# Autodesk Inventor assembly: Bari Cart
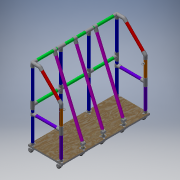
[picture p0: Inventor's stored thumbnail of the model, 180x180]
Saved by Autodesk Inventor 2018.2 (Build 222227000, 227)
## iProperties
Created: 2018-03-15
Part Number: Bari Cart
Document SubType Name: Assembly
Designer: owner
Author: owner
## Documents named in this file (20)
- Z:\The Pickle - 4 - Copy\Final Carts\Sax Cart\Bari Sax Cart.iam
- Z:\The Pickle - 4 - Copy\Final Carts\Sax Cart\Bari Plywood Base.ipt
- Z:\The Pickle - 4 - Copy\Final Carts\Stuff Used By All Carts\PVC Fittings (Formufit)\Wood Mount 1 Inch.ipt
- Z:\The Pickle - 4 - Copy\Final Carts\Stuff Used By All Carts\PVC Fittings (Formufit)\3-way 90 1 Inch.ipt
- Z:\The Pickle - 4 - Copy\Final Carts\Stuff Used By All Carts\PVC Fittings (Formufit)\45 Elbow 1 Inch.ipt
- Z:\The Pickle - 4 - Copy\Final Carts\Stuff Used By All Carts\PVC Fittings (Formufit)\Cross 1 Inch.ipt
- Z:\The Pickle - 4 - Copy\Final Carts\Stuff Used By All Carts\PVC Fittings (Formufit)\Formufit Pipe 1 Inch Flush Fittings.ipt
- Z:\The Pickle - 4 - Copy\Final Carts\Stuff Used By All Carts\PVC Fittings (Formufit)\Slip Tee 1 Inch.ipt
- Z:\The Pickle - 4 - Copy\Final Carts\Stuff Used By All Carts\PVC Fittings (Formufit)\Tee 1 Inch.ipt
- Z:\The Pickle - 4 - Copy\Final Carts\Sax Cart\Adjustable Elbow 1 Inch - Sax Angle.iam
- Z:\The Pickle - 4 - Copy\Final Carts\Sax Cart\Sax Pipe 1 (Tenor and Bari).ipt
- Z:\The Pickle - 4 - Copy\Final Carts\Sax Cart\Sax Pipe 2 (Tenor and Bari).ipt
- Z:\The Pickle - 4 - Copy\Final Carts\Sax Cart\Bari Sax Pipe 5.ipt
- Z:\The Pickle - 4 - Copy\Final Carts\Sax Cart\Bari Sax Pipe 4.ipt
- Z:\The Pickle - 4 - Copy\Final Carts\Sax Cart\Bari Sax Pipe 6.ipt
- Z:\The Pickle - 4 - Copy\Final Carts\Sax Cart\Bari Sax Pipe 7.ipt
- Z:\The Pickle - 4 - Copy\Final Carts\Sax Cart\Bari Sax Pipe OD - ID Adaptor.ipt
- Z:\The Pickle - 4 - Copy\Final Carts\Sax Cart\Bari Sax Wheel.ipt
- Z:\The Pickle - 4 - Copy\Final Carts\Sax Cart\Eyenut Screw.ipt
- Z:\The Pickle - 4 - Copy\Final Carts\Sax Cart\Eyenut.ipt
## Components (76 placed, 19 different names)
1. Bari Plywood Base:1 — Mate:1, Tangent:1, Tangent:2, Tangent:3, Mate:10, Mate:11, Mate:12, Flush:32, Flush:33, Flush:34, Mate:16, Tangent:4, Tangent:5, Flush:35
2. Wood Mount 1 Inch:1 — Mate:1, Tangent:1, Tangent:2, Tangent:3, Insert:1
3. Wood Mount 1 Inch:3 — Flush:3, Insert:6, Tangent:4
4. Wood Mount 1 Inch:4 — Flush:3, Flush:4, Insert:4, Tangent:5
5. Wood Mount 1 Inch:5 — Flush:5, Insert:3
6. Wood Mount 1 Inch:6 — Insert:2
7. Wood Mount 1 Inch:8 — Flush:4, Flush:5, Insert:5
8. 3-way 90 1 Inch:1 — Insert:18, Insert:21, Mate:8
9. 3-way 90 1 Inch:2 — Insert:35, Insert:37, Insert:39
10. 45 Elbow 1 Inch:1 — Insert:14, Mate:30
11. 45 Elbow 1 Inch:2 — Insert:42, Insert:43, Mate:27
12. 45 Elbow 1 Inch:3 — Insert:16, Insert:17
13. 45 Elbow 1 Inch:4 — Insert:40, Insert:41
14. Cross 1 Inch:1 — Insert:23, Insert:27, Insert:28
15. Cross 1 Inch:2 — Insert:30, Insert:31, Insert:33
16. Formufit Pipe 1 Inch Flush Fittings:1 — Insert:39, Insert:40
17. Formufit Pipe 1 Inch Flush Fittings:2 — Insert:17, Insert:18
18. Slip Tee 1 Inch:1 — Insert:12, Mate:2
19. Slip Tee 1 Inch:2 — Insert:47, Mate:3
20. Slip Tee 1 Inch:3 — Mate:6, Mate:9, Mate:15
21. Slip Tee 1 Inch:4 — Mate:5, Mate:7, Mate:9, Mate:14
22. Tee 1 Inch:1 — Insert:19, Insert:20, Insert:22
23. Tee 1 Inch:2 — Insert:36, Insert:38
24. Tee 1 Inch:3 — Insert:24, Insert:25, Insert:26
25. Tee 1 Inch:4 — Insert:29, Insert:32, Insert:34
26. Tee 1 Inch:5 — Insert:44, Insert:45, Insert:46, Mate:28
27. Tee 1 Inch:6 — Insert:10, Insert:11, Insert:13, Mate:31
28. Adjustable Elbow 1 Inch - Sax Angle:1 [sub-assembly] — Insert:53, Mate:15, Insert:56
29. Adjustable Elbow 1 Inch - Sax Angle:2 [sub-assembly] — Insert:51, Mate:13, Insert:54
30. Adjustable Elbow 1 Inch - Sax Angle:3 [sub-assembly] — Insert:52, Mate:14, Insert:55
31. Sax Pipe 1 (Tenor and Bari):1 — Insert:3, Insert:31
32. Sax Pipe 1 (Tenor and Bari):2 — Insert:4, Insert:38, Mate:3, Mate:23
33. Sax Pipe 1 (Tenor and Bari):3 — Insert:5, Insert:28
34. Sax Pipe 1 (Tenor and Bari):4 — Insert:20
35. Sax Pipe 1 (Tenor and Bari):5 — Insert:25
36. Sax Pipe 1 (Tenor and Bari):6 — Insert:32
37. Sax Pipe 1 (Tenor and Bari):7 — Insert:37, Mate:21, Mate:22
38. Sax Pipe 1 (Tenor and Bari):8 — Insert:2, Mate:2, Insert:19
39. Sax Pipe 2 (Tenor and Bari):1 — Insert:21, Insert:24, Mate:4
40. Sax Pipe 2 (Tenor and Bari):2 — Insert:26, Insert:29, Mate:5
41. Sax Pipe 2 (Tenor and Bari):3 — Insert:33, Insert:36
42. Sax Pipe 2 (Tenor and Bari):4 — Insert:34, Insert:35, Mate:6
43. Sax Pipe 2 (Tenor and Bari):5 — Insert:27, Insert:30
44. Sax Pipe 2 (Tenor and Bari):6 — Insert:22, Insert:23
45. Bari Sax Pipe 5:1 — Insert:11, Insert:12
46. Bari Sax Pipe 5:2 — Insert:46, Insert:47
47. Bari Sax Pipe 5:3 — Insert:1, Insert:10
48. Bari Sax Pipe 5:4 — Insert:6, Insert:45
49. Bari Sax Pipe 4:1 — Insert:54, Mate:17
50. Bari Sax Pipe 4:2 — Insert:55, Mate:18
51. Bari Sax Pipe 6:1 — Insert:16
52. Bari Sax Pipe 6:2 — Insert:41, Insert:42
53. Bari Sax Pipe 7:1 — Insert:13, Insert:14, Tangent:8, Tangent:9
54. Bari Sax Pipe 7:2 — Insert:43, Insert:44, Mate:20, Tangent:6, Tangent:7
55. Slip Tee 1 Inch:5 — Mate:4, Mate:7, Mate:8, Mate:13
56. Wood Mount 1 Inch:11 — Mate:10, Insert:50
57. Wood Mount 1 Inch:12 — Mate:11, Insert:49
58. Wood Mount 1 Inch:13 — Mate:12, Insert:48
59. Bari Sax Pipe OD - ID Adaptor:1 — Insert:48, Insert:53
60. Bari Sax Pipe OD - ID Adaptor:2 — Insert:50, Insert:51
61. Bari Sax Pipe OD - ID Adaptor:3 — Insert:49, Insert:52
62. Bari Sax Pipe 4:3 — Insert:56, Mate:19
63. Bari Sax Wheel:1 — Flush:6, Flush:10, Flush:15, Flush:22, Flush:32, Flush:33
64. Bari Sax Wheel:2 — Flush:6, Flush:7, Flush:11, Flush:16, Flush:22, Flush:23, Mate:17
65. Bari Sax Wheel:3 — Flush:7, Flush:8, Flush:12, Flush:17, Flush:23, Flush:24, Mate:18
66. Bari Sax Wheel:4 — Flush:8, Flush:9, Flush:13, Flush:18, Flush:24, Flush:25, Mate:19
67. Bari Sax Wheel:5 — Flush:9, Flush:19, Flush:25, Flush:35
68. Bari Sax Wheel:6 — Flush:14, Flush:19, Flush:27
69. Bari Sax Wheel:7 — Flush:13, Flush:14, Flush:18, Flush:26, Flush:27
70. Bari Sax Wheel:8 — Flush:12, Flush:17, Flush:21, Flush:26
71. Bari Sax Wheel:9 — Flush:11, Flush:16, Flush:20, Flush:21
72. Bari Sax Wheel:10 — Flush:10, Flush:15, Flush:20, Flush:34, Mate:16
73. Eyenut Screw:1 — Tangent:6, Mate:26, Mate:27, Mate:28
74. Eyenut:1 — Tangent:7, Mate:26
75. Eyenut Screw:2 — Mate:29, Tangent:9, Mate:30, Mate:31
76. Eyenut:2 — Mate:29, Tangent:8
## Relationships (121: Insert 52, Mate 31, Flush 29, Tangent 9)
- Flush:3: Wood Mount 1 Inch:3 ↔ Wood Mount 1 Inch:4
- Flush:4: Wood Mount 1 Inch:4 ↔ Wood Mount 1 Inch:8
- Flush:5: Wood Mount 1 Inch:5 ↔ Wood Mount 1 Inch:8
- Mate:1: Bari Plywood Base:1 ↔ Wood Mount 1 Inch:1
- Tangent:1: Bari Plywood Base:1 ↔ Wood Mount 1 Inch:1
- Tangent:2: Bari Plywood Base:1 ↔ Wood Mount 1 Inch:1
- Tangent:3: Bari Plywood Base:1 ↔ Wood Mount 1 Inch:1
- Insert:1: Wood Mount 1 Inch:1 ↔ Bari Sax Pipe 5:3
- Insert:2: Wood Mount 1 Inch:6 ↔ Sax Pipe 1 (Tenor and Bari):8
- Insert:3: Wood Mount 1 Inch:5 ↔ Sax Pipe 1 (Tenor and Bari):1
- Insert:4: Wood Mount 1 Inch:4 ↔ Sax Pipe 1 (Tenor and Bari):2
- Insert:5: Wood Mount 1 Inch:8 ↔ Sax Pipe 1 (Tenor and Bari):3
- Insert:6: Wood Mount 1 Inch:3 ↔ Bari Sax Pipe 5:4
- Insert:10: Tee 1 Inch:6 ↔ Bari Sax Pipe 5:3
- Insert:11: Tee 1 Inch:6 ↔ Bari Sax Pipe 5:1
- Insert:12: Slip Tee 1 Inch:1 ↔ Bari Sax Pipe 5:1
- Mate:2: Slip Tee 1 Inch:1 ↔ Sax Pipe 1 (Tenor and Bari):8
- Insert:13: Tee 1 Inch:6 ↔ Bari Sax Pipe 7:1
- Insert:14: 45 Elbow 1 Inch:1 ↔ Bari Sax Pipe 7:1
- Insert:16: 45 Elbow 1 Inch:3 ↔ Bari Sax Pipe 6:1
- Insert:17: 45 Elbow 1 Inch:3 ↔ Formufit Pipe 1 Inch Flush Fittings:2
- Insert:18: 3-way 90 1 Inch:1 ↔ Formufit Pipe 1 Inch Flush Fittings:2
- Insert:19: Tee 1 Inch:1 ↔ Sax Pipe 1 (Tenor and Bari):8
- Insert:20: Tee 1 Inch:1 ↔ Sax Pipe 1 (Tenor and Bari):4
- Insert:21: 3-way 90 1 Inch:1 ↔ Sax Pipe 2 (Tenor and Bari):1
- Insert:22: Tee 1 Inch:1 ↔ Sax Pipe 2 (Tenor and Bari):6
- Insert:23: Cross 1 Inch:1 ↔ Sax Pipe 2 (Tenor and Bari):6
- Insert:24: Tee 1 Inch:3 ↔ Sax Pipe 2 (Tenor and Bari):1
- Insert:25: Tee 1 Inch:3 ↔ Sax Pipe 1 (Tenor and Bari):5
- Insert:26: Tee 1 Inch:3 ↔ Sax Pipe 2 (Tenor and Bari):2
- Insert:27: Cross 1 Inch:1 ↔ Sax Pipe 2 (Tenor and Bari):5
- Insert:28: Cross 1 Inch:1 ↔ Sax Pipe 1 (Tenor and Bari):3
- Insert:29: Tee 1 Inch:4 ↔ Sax Pipe 2 (Tenor and Bari):2
- Insert:30: Cross 1 Inch:2 ↔ Sax Pipe 2 (Tenor and Bari):5
- Insert:31: Cross 1 Inch:2 ↔ Sax Pipe 1 (Tenor and Bari):1
- Insert:32: Tee 1 Inch:4 ↔ Sax Pipe 1 (Tenor and Bari):6
- Insert:33: Cross 1 Inch:2 ↔ Sax Pipe 2 (Tenor and Bari):3
- Insert:34: Tee 1 Inch:4 ↔ Sax Pipe 2 (Tenor and Bari):4
- Insert:35: 3-way 90 1 Inch:2 ↔ Sax Pipe 2 (Tenor and Bari):4
- Insert:36: Tee 1 Inch:2 ↔ Sax Pipe 2 (Tenor and Bari):3
- Insert:37: 3-way 90 1 Inch:2 ↔ Sax Pipe 1 (Tenor and Bari):7
- Insert:38: Tee 1 Inch:2 ↔ Sax Pipe 1 (Tenor and Bari):2
- Insert:39: 3-way 90 1 Inch:2 ↔ Formufit Pipe 1 Inch Flush Fittings:1
- Insert:40: 45 Elbow 1 Inch:4 ↔ Formufit Pipe 1 Inch Flush Fittings:1
- Insert:41: 45 Elbow 1 Inch:4 ↔ Bari Sax Pipe 6:2
- Insert:42: 45 Elbow 1 Inch:2 ↔ Bari Sax Pipe 6:2
- Insert:43: 45 Elbow 1 Inch:2 ↔ Bari Sax Pipe 7:2
- Insert:44: Tee 1 Inch:5 ↔ Bari Sax Pipe 7:2
- Insert:45: Tee 1 Inch:5 ↔ Bari Sax Pipe 5:4
- Insert:46: Tee 1 Inch:5 ↔ Bari Sax Pipe 5:2
- Insert:47: Slip Tee 1 Inch:2 ↔ Bari Sax Pipe 5:2
- Mate:3: Slip Tee 1 Inch:2 ↔ Sax Pipe 1 (Tenor and Bari):2
- Mate:4: Sax Pipe 2 (Tenor and Bari):1 ↔ Slip Tee 1 Inch:5
- Mate:5: Slip Tee 1 Inch:4 ↔ Sax Pipe 2 (Tenor and Bari):2
- Mate:6: Slip Tee 1 Inch:3 ↔ Sax Pipe 2 (Tenor and Bari):4
- Mate:7 (225.425 mm): Slip Tee 1 Inch:4 ↔ Slip Tee 1 Inch:5
- Mate:8 (246.0625 mm): 3-way 90 1 Inch:1 ↔ Slip Tee 1 Inch:5
- Mate:9 (225.425 mm): Slip Tee 1 Inch:3 ↔ Slip Tee 1 Inch:4
- Mate:10: Bari Plywood Base:1 ↔ Wood Mount 1 Inch:11
- Mate:11: Bari Plywood Base:1 ↔ Wood Mount 1 Inch:12
- Mate:12: Bari Plywood Base:1 ↔ Wood Mount 1 Inch:13
- Insert:48: Wood Mount 1 Inch:13 ↔ Bari Sax Pipe OD - ID Adaptor:1
- Insert:49: Wood Mount 1 Inch:12 ↔ Bari Sax Pipe OD - ID Adaptor:3
- Insert:50: Wood Mount 1 Inch:11 ↔ Bari Sax Pipe OD - ID Adaptor:2
- Insert:51: Adjustable Elbow 1 Inch - Sax Angle:2 ↔ Bari Sax Pipe OD - ID Adaptor:2
- Insert:52: Adjustable Elbow 1 Inch - Sax Angle:3 ↔ Bari Sax Pipe OD - ID Adaptor:3
- Insert:53: Adjustable Elbow 1 Inch - Sax Angle:1 ↔ Bari Sax Pipe OD - ID Adaptor:1
- Mate:13: Adjustable Elbow 1 Inch - Sax Angle:2 ↔ Slip Tee 1 Inch:5
- Mate:14: Slip Tee 1 Inch:4 ↔ Adjustable Elbow 1 Inch - Sax Angle:3
- Mate:15: Slip Tee 1 Inch:3 ↔ Adjustable Elbow 1 Inch - Sax Angle:1
- Insert:54: Adjustable Elbow 1 Inch - Sax Angle:2 ↔ Bari Sax Pipe 4:1
- Insert:55: Adjustable Elbow 1 Inch - Sax Angle:3 ↔ Bari Sax Pipe 4:2
- Insert:56: Adjustable Elbow 1 Inch - Sax Angle:1 ↔ Bari Sax Pipe 4:3
- Flush:6: Bari Sax Wheel:1 ↔ Bari Sax Wheel:2
- Flush:7: Bari Sax Wheel:2 ↔ Bari Sax Wheel:3
- Flush:8: Bari Sax Wheel:3 ↔ Bari Sax Wheel:4
- Flush:9: Bari Sax Wheel:4 ↔ Bari Sax Wheel:5
- Flush:10: Bari Sax Wheel:1 ↔ Bari Sax Wheel:10
- Flush:11: Bari Sax Wheel:2 ↔ Bari Sax Wheel:9
- Flush:12: Bari Sax Wheel:3 ↔ Bari Sax Wheel:8
- Flush:13: Bari Sax Wheel:4 ↔ Bari Sax Wheel:7
- Flush:14: Bari Sax Wheel:6 ↔ Bari Sax Wheel:7
- Flush:15: Bari Sax Wheel:1 ↔ Bari Sax Wheel:10
- Flush:16: Bari Sax Wheel:2 ↔ Bari Sax Wheel:9
- Flush:17: Bari Sax Wheel:3 ↔ Bari Sax Wheel:8
- Flush:18: Bari Sax Wheel:4 ↔ Bari Sax Wheel:7
- Flush:19: Bari Sax Wheel:5 ↔ Bari Sax Wheel:6
- Flush:20: Bari Sax Wheel:9 ↔ Bari Sax Wheel:10
- Flush:21: Bari Sax Wheel:8 ↔ Bari Sax Wheel:9
- Flush:22: Bari Sax Wheel:1 ↔ Bari Sax Wheel:2
- Flush:23: Bari Sax Wheel:2 ↔ Bari Sax Wheel:3
- Flush:24: Bari Sax Wheel:3 ↔ Bari Sax Wheel:4
- Flush:25: Bari Sax Wheel:4 ↔ Bari Sax Wheel:5
- Flush:26: Bari Sax Wheel:7 ↔ Bari Sax Wheel:8
- Flush:27: Bari Sax Wheel:6 ↔ Bari Sax Wheel:7
- Flush:32: Bari Plywood Base:1 ↔ Bari Sax Wheel:1
- Flush:33: Bari Plywood Base:1 ↔ Bari Sax Wheel:1
- Flush:34: Bari Plywood Base:1 ↔ Bari Sax Wheel:10
- Mate:16: Bari Plywood Base:1 ↔ Bari Sax Wheel:10
- Mate:17 (-22.225 mm): Bari Sax Pipe 4:1 ↔ Bari Sax Wheel:2
- Mate:18 (-22.225 mm): Bari Sax Pipe 4:2 ↔ Bari Sax Wheel:3
- Mate:19 (-22.225 mm): Bari Sax Pipe 4:3 ↔ Bari Sax Wheel:4
- Tangent:4: Bari Plywood Base:1 ↔ Wood Mount 1 Inch:3
- Tangent:5: Bari Plywood Base:1 ↔ Wood Mount 1 Inch:4
- Flush:35: Bari Plywood Base:1 ↔ Bari Sax Wheel:5
- Mate:20: Bari Sax Pipe 7:2
- Mate:21: Sax Pipe 1 (Tenor and Bari):7
- Mate:22: Sax Pipe 1 (Tenor and Bari):7
- Mate:23: Sax Pipe 1 (Tenor and Bari):2
- Mate:24
- Mate:25
- Tangent:6: Bari Sax Pipe 7:2 ↔ Eyenut Screw:1
- Tangent:7: Bari Sax Pipe 7:2 ↔ Eyenut:1
- Mate:26: Eyenut Screw:1 ↔ Eyenut:1
- Mate:27 (38.1 mm): 45 Elbow 1 Inch:2 ↔ Eyenut Screw:1
- Mate:28 (-50.8 mm): Tee 1 Inch:5 ↔ Eyenut Screw:1
- Mate:29: Eyenut Screw:2 ↔ Eyenut:2
- Tangent:8: Bari Sax Pipe 7:1 ↔ Eyenut:2
- Tangent:9: Bari Sax Pipe 7:1 ↔ Eyenut Screw:2
- Mate:30 (38.1 mm): 45 Elbow 1 Inch:1 ↔ Eyenut Screw:2
- Mate:31 (-50.8 mm): Tee 1 Inch:6 ↔ Eyenut Screw:2
